# Autodesk Inventor assembly: robot
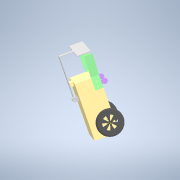
[picture p0: Inventor's stored thumbnail of the model, 180x180]
Saved by Autodesk Inventor 2020 (Build 240168000, 168)
## iProperties
Created: 2023-01-13
Part Number: robot
Document SubType Name: Assembly
Designer: hugoG
Author: hugoG
## Documents named in this file (7)
- D:\cours ensta\3A\IG\robot.iam
- D:\cours ensta\3A\IG\corps.ipt
- D:\cours ensta\3A\IG\wheel.ipt
- D:\cours ensta\3A\IG\ramasse.ipt
- D:\cours ensta\3A\IG\pelle.ipt
- D:\cours ensta\3A\IG\support pelle.ipt
- D:\cours ensta\3A\IG\Assembly2.iam
## Components (10 placed, 6 different names)
1. corps:1 — Mate:1, Mate:2, Mate:3, Mate:4, Mate:5, Mate:6, Mate:7, Mate:8, Mate:9, Mate:10, Mate:11, Mate:12, Mate:13, Mate:14, Mate:15, Mate:16, Mate:20, Mate:21, Mate:22, Mate:23, Mate:24, Mate:25
2. wheel:1 — Mate:1, Mate:2
3. wheel:2 — Mate:3, Mate:4
4. ramasse:1 — Mate:5, Mate:6, Mate:7
5. ramasse:2 — Mate:8, Mate:9, Mate:10
6. pelle:1 — Mate:18, Mate:19
7. support pelle:1 — Mate:12, Mate:15, Mate:16, Mate:18, Mate:19
8. support pelle:2 — Mate:11, Mate:13, Mate:14
9. Assembly2:1 [sub-assembly] — Mate:21, Mate:24, Mate:25
10. Assembly2:2 [sub-assembly] — Mate:20, Mate:22, Mate:23
## Relationships (24: Mate 24)
- Mate:1: corps:1 ↔ wheel:1
- Mate:2: corps:1 ↔ wheel:1
- Mate:3: corps:1 ↔ wheel:2
- Mate:4: corps:1 ↔ wheel:2
- Mate:5: corps:1 ↔ ramasse:1
- Mate:6: corps:1 ↔ ramasse:1
- Mate:7: corps:1 ↔ ramasse:1
- Mate:8: corps:1 ↔ ramasse:2
- Mate:9: corps:1 ↔ ramasse:2
- Mate:10: corps:1 ↔ ramasse:2
- Mate:11: corps:1 ↔ support pelle:2
- Mate:12: corps:1 ↔ support pelle:1
- Mate:13: corps:1 ↔ support pelle:2
- Mate:14: corps:1 ↔ support pelle:2
- Mate:15: corps:1 ↔ support pelle:1
- Mate:16: corps:1 ↔ support pelle:1
- Mate:18: pelle:1 ↔ support pelle:1
- Mate:19: pelle:1 ↔ support pelle:1
- Mate:20: corps:1 ↔ Assembly2:2
- Mate:21: corps:1 ↔ Assembly2:1
- Mate:22: corps:1 ↔ Assembly2:2
- Mate:23: corps:1 ↔ Assembly2:2
- Mate:24: corps:1 ↔ Assembly2:1
- Mate:25: corps:1 ↔ Assembly2:1
